# Autodesk Inventor assembly: Front Left Wheel Hub Assemby
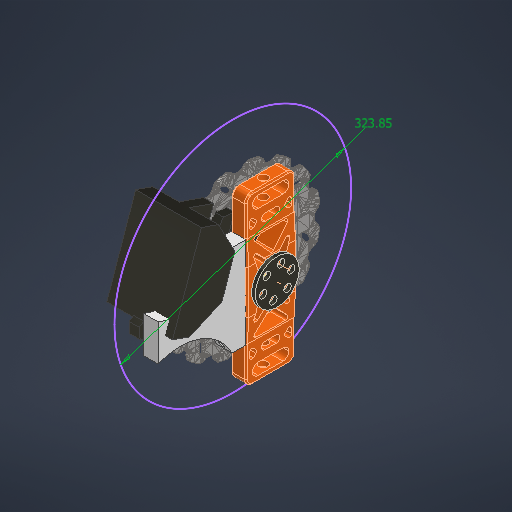
[picture p0: Inventor's stored thumbnail of the model, 512x512]
Saved by Autodesk Inventor 2026.1 (Build 301233000, 233)
## iProperties
Created: 2026-06-24
Part Number: Front Left Wheel Hub Assemby
Document SubType Name: Assembly
Designer: share
Author: share
## Documents named in this file (7)
- C:\Users\share\OneDrive\Documents\Personal Projects\GOGO Kart\CAD\GOGO_KART_FSAE\Suspension\Upright Assembly\Front Left Wheel Hub Assemby.iam
- C:\Users\share\OneDrive\Documents\Personal Projects\GOGO Kart\CAD\GOGO_KART_FSAE\Suspension\Upright Assembly\Front Upright.ipt
- C:\Users\share\OneDrive\Documents\Personal Projects\GOGO Kart\CAD\GOGO_KART_FSAE\Drivetrain\Rear_Wheel_Hub_Assembly.iam
- C:\Users\share\OneDrive\Documents\Personal Projects\GOGO Kart\CAD\GOGO_KART_FSAE\Suspension\Upright Assembly\Arashi Rear Brake Disc Rotors.ipt
- C:\Users\share\OneDrive\Documents\Personal Projects\GOGO Kart\CAD\GOGO_KART_FSAE\Suspension\Upright Assembly\2385K101_Angular Contact Single Row Ball Bearing.ipt
- C:\Users\share\OneDrive\Documents\Personal Projects\GOGO Kart\CAD\GOGO_KART_FSAE\Suspension\Upright Assembly\Caliper Bracket Mount V2.ipt
- C:\Users\share\OneDrive\Documents\Personal Projects\GOGO Kart\CAD\GOGO_KART_FSAE\Suspension\Upright Assembly\F3 Front Caliper Bracket.ipt
## Components (7 placed, 6 different names)
1. Front Upright:1 — Flush:1, Flush:2, Flush:3, Mate:1, Insert:5, Insert:6, Insert:8, Insert:9
2. Rear_Wheel_Hub_Assembly:1 [sub-assembly] — Mate:1, Insert:3, Insert:4, Insert:7
3. Arashi Rear Brake Disc Rotors:1 — Insert:3, Insert:4
4. 2385K101_Angular Contact Single Row Ball Bearing:1 — Insert:6, Insert:7
5. 2385K101_Angular Contact Single Row Ball Bearing:2 — Insert:5
6. Caliper Bracket Mount V2:1 — Insert:8, Insert:9, Insert:10, Insert:11
7. F3 Front Caliper Bracket:1 — Insert:10, Insert:11
## Relationships (13: Insert 9, Flush 3, Mate 1)
- Flush:1: Front Upright:1
- Flush:2: Front Upright:1
- Flush:3: Front Upright:1
- Mate:1: Front Upright:1 ↔ Rear_Wheel_Hub_Assembly:1
- Insert:3: Rear_Wheel_Hub_Assembly:1 ↔ Arashi Rear Brake Disc Rotors:1
- Insert:4: Rear_Wheel_Hub_Assembly:1 ↔ Arashi Rear Brake Disc Rotors:1
- Insert:5: Front Upright:1 ↔ 2385K101_Angular Contact Single Row Ball Bearing:2
- Insert:6: Front Upright:1 ↔ 2385K101_Angular Contact Single Row Ball Bearing:1
- Insert:7: Rear_Wheel_Hub_Assembly:1 ↔ 2385K101_Angular Contact Single Row Ball Bearing:1
- Insert:8: Front Upright:1 ↔ Caliper Bracket Mount V2:1
- Insert:9: Front Upright:1 ↔ Caliper Bracket Mount V2:1
- Insert:10: Caliper Bracket Mount V2:1 ↔ F3 Front Caliper Bracket:1
- Insert:11: Caliper Bracket Mount V2:1 ↔ F3 Front Caliper Bracket:1
